# Autodesk Inventor assembly: Weight Applier for Modules v3
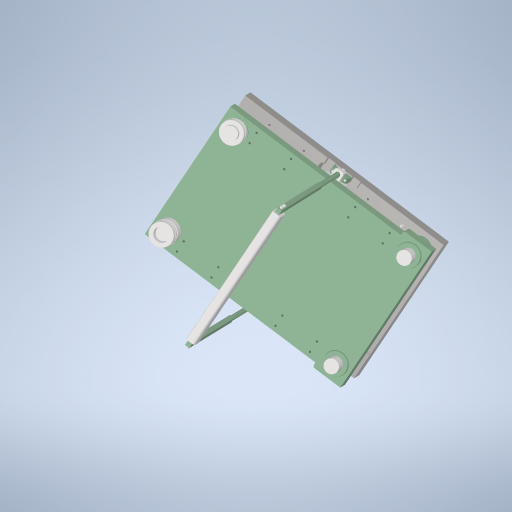
[picture p0: Inventor's stored thumbnail of the model, 512x512]
Saved by Autodesk Inventor 2023 (Build 270158000, 158)
## iProperties
Created: 2023-01-04
Part Number: Weight Applier for Modules v3
Document SubType Name: Assembly
Designer: Hayden Swanson
Author: Hayden Swanson
## Documents named in this file (13)
- C:\Users\Hayden Swanson\UNLAssemblyProject\Hardware\ETL\Module Assembly\WAM_v3\Weight Applier for Modules v3.iam
- C:\Users\Hayden Swanson\UNLAssemblyProject\Hardware\ETL\Module Assembly\Tamale Assembly Plate V3\Tamale Assembly Plate Assembly V3.iam
- C:\Users\Hayden Swanson\UNLAssemblyProject\Hardware\ETL\Module Assembly\WAM_v3\Rod.ipt
- C:\Users\Hayden Swanson\UNLAssemblyProject\Hardware\ETL\Module Assembly\WAM_v3\Weight Frame Top.ipt
- C:\Users\Hayden Swanson\UNLAssemblyProject\Hardware\ETL\Module Assembly\WAM_v3\Weight Frame.ipt
- C:\Users\Hayden Swanson\UNLAssemblyProject\Hardware\ETL\Module Assembly\WAM_v3\90272A972_Zinc-Plated Steel Pan Head Phillips Screw.ipt
- C:\Users\Hayden Swanson\UNLAssemblyProject\Hardware\ETL\Module Assembly\WAM_v3\90044A111_Black-Oxide Alloy Steel Socket Head Screw.ipt
- C:\Users\Hayden Swanson\UNLAssemblyProject\Hardware\ETL\Module Assembly\WAM_v3\handle.ipt
- C:\Users\Hayden Swanson\UNLAssemblyProject\Hardware\ETL\Module Assembly\WAM_v3\handle handle.ipt
- C:\Users\Hayden Swanson\UNLAssemblyProject\Hardware\ETL\Module Assembly\WAM_v3\9533T5_Self-Aligning Linear Sleeve Bearing.ipt
- C:\Users\Hayden Swanson\UNLAssemblyProject\Hardware\ETL\Module Assembly\WAM_v3\LockMechanism_v3.iam
- C:\Users\Hayden Swanson\UNLAssemblyProject\Hardware\ETL\Module Assembly\WAM_v3\91590A137_External Retaining Ring.ipt
- C:\Users\Hayden Swanson\UNLAssemblyProject\Hardware\ETL\Module Assembly\WAM_v3\9634K37_Extension Spring Stud Anchor.ipt
## Components (36 placed, 12 different names)
1. Tamale Assembly Plate Assembly V3:1 [sub-assembly] — Mate:1, Mate:75, Mate:85
2. Weight Frame:1 — Mate:1, Mate:75, Mate:85, Mate:111, Mate:120, Mate:127, Mate:128, Mate:129, Mate:130, Mate:131, Mate:132, Mate:133, Mate:134, Mate:135, Mate:136, Mate:137, Mate:138, Mate:139, Mate:140, Mate:141, Mate:142, Mate:160, Mate:161, Mate:162, Mate:163, Mate:164, Mate:165, Mate:166, Mate:167, Mate:170, Mate:173, Mate:183, Mate:184, Mate:189, Mate:191
3. Weight Frame Top:2 — Mate:113, Mate:122, Mate:180, Mate:181, Mate:182, Mate:192
4. handle:1 — Mate:91, Mate:92, Mate:150, Mate:152, Mate:155, Mate:156, Mate:157, Mate:174
5. handle:2 — Mate:93, Mate:94, Mate:151, Mate:153, Mate:154, Mate:175
6. handle handle:1 — Mate:150, Mate:151, Mate:152, Mate:157
7. 90044A111_Black-Oxide Alloy Steel Socket Head Screw:13 — Mate:91, Mate:156
8. 90044A111_Black-Oxide Alloy Steel Socket Head Screw:14 — Mate:92, Mate:155
9. 90044A111_Black-Oxide Alloy Steel Socket Head Screw:15 — Mate:93, Mate:154
10. 90044A111_Black-Oxide Alloy Steel Socket Head Screw:16 — Mate:94, Mate:153
11. Rod:1 — Mate:111, Mate:113, Mate:124, Mate:186
12. Rod:4 — Mate:120, Mate:122, Mate:123, Mate:185
13. 9533T5_Self-Aligning Linear Sleeve Bearing:1 — Mate:123
14. 9533T5_Self-Aligning Linear Sleeve Bearing:2 — Mate:124, Mate:176, Mate:177, Mate:178, Mate:179
15. 9533T5_Self-Aligning Linear Sleeve Bearing:3 — Mate:187
16. 90272A972_Zinc-Plated Steel Pan Head Phillips Screw:1 — Mate:166, Mate:167, Mate:187, Mate:188
17. 90272A972_Zinc-Plated Steel Pan Head Phillips Screw:2 — Mate:160, Mate:161, Mate:190
18. 90272A972_Zinc-Plated Steel Pan Head Phillips Screw:3 — Mate:162, Mate:163, Mate:185
19. 90044A111_Black-Oxide Alloy Steel Socket Head Screw:17 — Mate:127, Mate:132
20. 90044A111_Black-Oxide Alloy Steel Socket Head Screw:18 — Mate:129, Mate:131, Mate:169
21. 90044A111_Black-Oxide Alloy Steel Socket Head Screw:19 — Mate:130, Mate:133
22. 90044A111_Black-Oxide Alloy Steel Socket Head Screw:20 — Mate:128, Mate:134, Mate:168
23. 90044A111_Black-Oxide Alloy Steel Socket Head Screw:21 — Mate:135, Mate:141
24. 90044A111_Black-Oxide Alloy Steel Socket Head Screw:22 — Mate:136, Mate:142, Mate:171
25. 90044A111_Black-Oxide Alloy Steel Socket Head Screw:23 — Mate:137, Mate:140, Mate:172
26. 90044A111_Black-Oxide Alloy Steel Socket Head Screw:24 — Mate:138, Mate:139
27. 90272A972_Zinc-Plated Steel Pan Head Phillips Screw:4 — Mate:164, Mate:165, Mate:186
28. LockMechanism_v3:1 [sub-assembly] — Mate:168, Mate:169, Mate:170, Mate:175
29. LockMechanism_v3:2 [sub-assembly] — Mate:171, Mate:172, Mate:173, Mate:174
30. 91590A137_External Retaining Ring:1 — Mate:176, Mate:177
31. 91590A137_External Retaining Ring:2 — Mate:178, Mate:179, Mate:180
32. 9634K37_Extension Spring Stud Anchor:1 — Mate:181, Mate:182
33. 9634K37_Extension Spring Stud Anchor:2 — Mate:183, Mate:184
34. Rod:5 — Mate:188, Mate:189
35. Rod:6 — Mate:190, Mate:191
36. 9533T5_Self-Aligning Linear Sleeve Bearing:4 — Mate:192
## Relationships (70: Mate 70)
- Mate:1: Tamale Assembly Plate Assembly V3:1 ↔ Weight Frame:1
- Mate:75: Tamale Assembly Plate Assembly V3:1 ↔ Weight Frame:1
- Mate:85: Tamale Assembly Plate Assembly V3:1 ↔ Weight Frame:1
- Mate:91: handle:1 ↔ 90044A111_Black-Oxide Alloy Steel Socket Head Screw:13
- Mate:92: handle:1 ↔ 90044A111_Black-Oxide Alloy Steel Socket Head Screw:14
- Mate:93: handle:2 ↔ 90044A111_Black-Oxide Alloy Steel Socket Head Screw:15
- Mate:94: handle:2 ↔ 90044A111_Black-Oxide Alloy Steel Socket Head Screw:16
- Mate:111: Weight Frame:1 ↔ Rod:1
- Mate:113: Weight Frame Top:2 ↔ Rod:1
- Mate:120: Weight Frame:1 ↔ Rod:4
- Mate:122: Weight Frame Top:2 ↔ Rod:4
- Mate:123: Rod:4 ↔ 9533T5_Self-Aligning Linear Sleeve Bearing:1
- Mate:124: Rod:1 ↔ 9533T5_Self-Aligning Linear Sleeve Bearing:2
- Mate:127: Weight Frame:1 ↔ 90044A111_Black-Oxide Alloy Steel Socket Head Screw:17
- Mate:128: Weight Frame:1 ↔ 90044A111_Black-Oxide Alloy Steel Socket Head Screw:20
- Mate:129: Weight Frame:1 ↔ 90044A111_Black-Oxide Alloy Steel Socket Head Screw:18
- Mate:130: Weight Frame:1 ↔ 90044A111_Black-Oxide Alloy Steel Socket Head Screw:19
- Mate:131: Weight Frame:1 ↔ 90044A111_Black-Oxide Alloy Steel Socket Head Screw:18
- Mate:132: Weight Frame:1 ↔ 90044A111_Black-Oxide Alloy Steel Socket Head Screw:17
- Mate:133: Weight Frame:1 ↔ 90044A111_Black-Oxide Alloy Steel Socket Head Screw:19
- Mate:134: Weight Frame:1 ↔ 90044A111_Black-Oxide Alloy Steel Socket Head Screw:20
- Mate:135: Weight Frame:1 ↔ 90044A111_Black-Oxide Alloy Steel Socket Head Screw:21
- Mate:136: Weight Frame:1 ↔ 90044A111_Black-Oxide Alloy Steel Socket Head Screw:22
- Mate:137: Weight Frame:1 ↔ 90044A111_Black-Oxide Alloy Steel Socket Head Screw:23
- Mate:138: Weight Frame:1 ↔ 90044A111_Black-Oxide Alloy Steel Socket Head Screw:24
- Mate:139: Weight Frame:1 ↔ 90044A111_Black-Oxide Alloy Steel Socket Head Screw:24
- Mate:140: Weight Frame:1 ↔ 90044A111_Black-Oxide Alloy Steel Socket Head Screw:23
- Mate:141: Weight Frame:1 ↔ 90044A111_Black-Oxide Alloy Steel Socket Head Screw:21
- Mate:142: Weight Frame:1 ↔ 90044A111_Black-Oxide Alloy Steel Socket Head Screw:22
- Mate:150: handle:1 ↔ handle handle:1
- Mate:151: handle:2 ↔ handle handle:1
- Mate:152: handle:1 ↔ handle handle:1
- Mate:153: handle:2 ↔ 90044A111_Black-Oxide Alloy Steel Socket Head Screw:16
- Mate:154: handle:2 ↔ 90044A111_Black-Oxide Alloy Steel Socket Head Screw:15
- Mate:155: handle:1 ↔ 90044A111_Black-Oxide Alloy Steel Socket Head Screw:14
- Mate:156: handle:1 ↔ 90044A111_Black-Oxide Alloy Steel Socket Head Screw:13
- Mate:157: handle:1 ↔ handle handle:1
- Mate:160: Weight Frame:1 ↔ 90272A972_Zinc-Plated Steel Pan Head Phillips Screw:2
- Mate:161: Weight Frame:1 ↔ 90272A972_Zinc-Plated Steel Pan Head Phillips Screw:2
- Mate:162: Weight Frame:1 ↔ 90272A972_Zinc-Plated Steel Pan Head Phillips Screw:3
- Mate:163: Weight Frame:1 ↔ 90272A972_Zinc-Plated Steel Pan Head Phillips Screw:3
- Mate:164: Weight Frame:1 ↔ 90272A972_Zinc-Plated Steel Pan Head Phillips Screw:4
- Mate:165: Weight Frame:1 ↔ 90272A972_Zinc-Plated Steel Pan Head Phillips Screw:4
- Mate:166: Weight Frame:1 ↔ 90272A972_Zinc-Plated Steel Pan Head Phillips Screw:1
- Mate:167: Weight Frame:1 ↔ 90272A972_Zinc-Plated Steel Pan Head Phillips Screw:1
- Mate:168: 90044A111_Black-Oxide Alloy Steel Socket Head Screw:20 ↔ LockMechanism_v3:1
- Mate:169: 90044A111_Black-Oxide Alloy Steel Socket Head Screw:18 ↔ LockMechanism_v3:1
- Mate:170: Weight Frame:1 ↔ LockMechanism_v3:1
- Mate:171: 90044A111_Black-Oxide Alloy Steel Socket Head Screw:22 ↔ LockMechanism_v3:2
- Mate:172: 90044A111_Black-Oxide Alloy Steel Socket Head Screw:23 ↔ LockMechanism_v3:2
- Mate:173: Weight Frame:1 ↔ LockMechanism_v3:2
- Mate:174: handle:1 ↔ LockMechanism_v3:2
- Mate:175: handle:2 ↔ LockMechanism_v3:1
- Mate:176: 9533T5_Self-Aligning Linear Sleeve Bearing:2 ↔ 91590A137_External Retaining Ring:1
- Mate:177: 9533T5_Self-Aligning Linear Sleeve Bearing:2 ↔ 91590A137_External Retaining Ring:1
- Mate:178: 9533T5_Self-Aligning Linear Sleeve Bearing:2 ↔ 91590A137_External Retaining Ring:2
- Mate:179: 9533T5_Self-Aligning Linear Sleeve Bearing:2 ↔ 91590A137_External Retaining Ring:2
- Mate:180: Weight Frame Top:2 ↔ 91590A137_External Retaining Ring:2
- Mate:181: Weight Frame Top:2 ↔ 9634K37_Extension Spring Stud Anchor:1
- Mate:182: Weight Frame Top:2 ↔ 9634K37_Extension Spring Stud Anchor:1
- Mate:183: Weight Frame:1 ↔ 9634K37_Extension Spring Stud Anchor:2
- Mate:184: Weight Frame:1 ↔ 9634K37_Extension Spring Stud Anchor:2
- Mate:185: Rod:4 ↔ 90272A972_Zinc-Plated Steel Pan Head Phillips Screw:3
- Mate:186: Rod:1 ↔ 90272A972_Zinc-Plated Steel Pan Head Phillips Screw:4
- Mate:187: 9533T5_Self-Aligning Linear Sleeve Bearing:3 ↔ 90272A972_Zinc-Plated Steel Pan Head Phillips Screw:1
- Mate:188: 90272A972_Zinc-Plated Steel Pan Head Phillips Screw:1 ↔ Rod:5
- Mate:189: Weight Frame:1 ↔ Rod:5
- Mate:190: 90272A972_Zinc-Plated Steel Pan Head Phillips Screw:2 ↔ Rod:6
- Mate:191: Weight Frame:1 ↔ Rod:6
- Mate:192: Weight Frame Top:2 ↔ 9533T5_Self-Aligning Linear Sleeve Bearing:4
